# Autodesk Inventor assembly: assemby
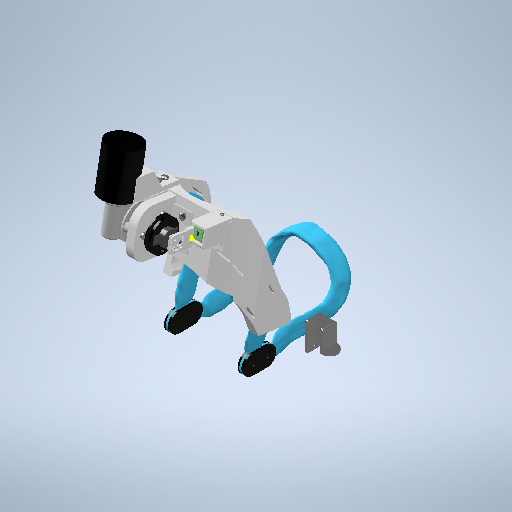
[picture p0: Inventor's stored thumbnail of the model, 512x512]
Saved by Autodesk Inventor 2025.2 (Build 292293000, 293)
## iProperties
Created: 2025-01-03
Part Number: assemby
Document SubType Name: Assembly
Designer: turbo
Author: turbo
## Documents named in this file (8)
- C:\Users\email\Desktop\Projects\Capstone\4TB6\CAD_Model\thigh_mount\assemby.iam
- C:\Users\email\Desktop\Projects\Capstone\4TB6\CAD_Model\thigh_mount\thigh.ipt
- C:\Users\email\Desktop\Projects\Capstone\4TB6\CAD_Model\thigh_mount\shin.ipt
- C:\Users\email\Desktop\Projects\Capstone\4TB6\CAD_Model\thigh_mount\hinge.ipt
- C:\Users\email\Desktop\Projects\Capstone\4TB6\CAD_Model\thigh_mount\rivet.ipt
- C:\Users\email\Desktop\Projects\Capstone\4TB6\CAD_Model\thigh_mount\thighmountassembly.iam
- C:\Users\email\Desktop\Projects\Capstone\4TB6\CAD_Model\thigh_mount\imu_mount.ipt
- C:\Shared\alex-bartella-schoolwork\4z03\final\final\Part1.ipt
## Components (13 placed, 7 different names)
1. thigh:1 — Mate:1, Mate:3, Mate:4, Rotation:1, Angle:2, Mate:8, Mate:9, Mate:11, Flush:1, Flush:2, Flush:3
2. shin:1 — Mate:2, Mate:5, Rotation:1, Mate:10, Mate:12, Mate:13, Mate:14, Angle:3
3. hinge:1 — Mate:3, Mate:4, Mate:5, Angle:1, Angle:2, Mate:6, Mate:7
4. hinge:2 — Mate:6, Mate:7, Mate:8, Insert:3, Insert:4
5. hinge:3 — Mate:9, Mate:10, Mate:13, Insert:1, Insert:2
6. hinge:4 — Mate:11, Mate:12, Mate:14, Angle:3
7. rivet:1 — Insert:1
8. rivet:2 — Insert:3
9. rivet:3 — Insert:4
10. rivet:4 — Insert:2
11. thighmountassembly:1 [sub-assembly] — Flush:1, Flush:2, Flush:3
12. imu_mount:1
13. Part1:1
## Relationships (25: Mate 14, Insert 4, Angle 3, Flush 3, RelateRotation 1)
- Mate:1: thigh:1
- Mate:2: shin:1
- Mate:3: thigh:1 ↔ hinge:1
- Mate:4: thigh:1 ↔ hinge:1
- Mate:5: shin:1 ↔ hinge:1
- Angle:1 (0 deg): hinge:1
- Rotation:1 [RelateRotation] (1 ul): thigh:1 ↔ shin:1
- Angle:2 (-20 deg): thigh:1 ↔ hinge:1
- Mate:6: hinge:1 ↔ hinge:2
- Mate:7: hinge:1 ↔ hinge:2
- Mate:8: thigh:1 ↔ hinge:2
- Mate:9: thigh:1 ↔ hinge:3
- Mate:10: shin:1 ↔ hinge:3
- Mate:11: thigh:1 ↔ hinge:4
- Mate:12: shin:1 ↔ hinge:4
- Mate:13: shin:1 ↔ hinge:3
- Mate:14: shin:1 ↔ hinge:4
- Insert:1: hinge:3 ↔ rivet:1
- Insert:2: hinge:3 ↔ rivet:4
- Insert:3: hinge:2 ↔ rivet:2
- Insert:4: hinge:2 ↔ rivet:3
- Angle:3 (88.82 deg): shin:1 ↔ hinge:4
- Flush:1: thigh:1 ↔ thighmountassembly:1
- Flush:2: thigh:1 ↔ thighmountassembly:1
- Flush:3: thigh:1 ↔ thighmountassembly:1
